# Autodesk Inventor assembly: printer
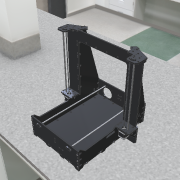
[picture p0: Inventor's stored thumbnail of the model, 180x180]
Saved by Autodesk Inventor 2014 (Build 180170000, 170)
## iProperties
Created: 2014-01-09
Part Number: printer
Document SubType Name: Assembly
Designer: buben
Author: buben
## Documents named in this file (21)
- C:\Users\buben\Documents\GitHub\bacon\inventor files\assemblies\printer.iam
- C:\Users\buben\Documents\GitHub\bacon\inventor files\printer parts\brace_left.ipt
- C:\Users\buben\Documents\GitHub\bacon\inventor files\printer parts\bottom.ipt
- C:\Users\buben\Documents\GitHub\bacon\inventor files\printer parts\brace_right.ipt
- C:\Users\buben\Documents\GitHub\bacon\inventor files\printer parts\front.ipt
- C:\Users\buben\Documents\GitHub\bacon\inventor files\printer parts\back.ipt
- C:\Users\buben\Documents\GitHub\bacon\inventor files\printer parts\frame.ipt
- C:\Users\buben\Documents\GitHub\bacon\inventor files\printer parts\z_motor_brace.ipt
- C:\Users\buben\Documents\GitHub\bacon\inventor files\printer parts\z_motor_mount.ipt
- C:\Users\buben\Documents\GitHub\bacon\inventor files\printer parts\y_axis_cap.ipt
- C:\Users\buben\Documents\GitHub\bacon\inventor files\printer parts\z_rod_stopper_bottom.ipt
- C:\Users\buben\Documents\GitHub\bacon\inventor files\3rd party components\nema_17_stepper\Imported Components\NEMA 17\NEMA 17.iam
- C:\Users\buben\Documents\GitHub\bacon\inventor files\utils\z_axis_rod.ipt
- C:\Users\buben\Documents\GitHub\bacon\inventor files\utils\z_threaded_rod.ipt
- C:\Users\buben\Documents\GitHub\bacon\inventor files\utils\y_axis_rod.ipt
- C:\Users\buben\Documents\GitHub\bacon\inventor files\printer parts\z_axis_top.ipt
- C:\Users\buben\Documents\GitHub\bacon\inventor files\printer parts\z_axis_top_cap.ipt
- C:\Users\buben\Documents\GitHub\bacon\inventor files\printer parts\frame_brace_top.ipt
- C:\Users\buben\Documents\GitHub\bacon\inventor files\utils\washer_m4.ipt
- C:\Users\buben\Documents\Inventor\Content Center Files\R2014\en-US\ISO 4762(2)\ISO 4762 - M4 x 20ISO.ipt
- C:\Users\buben\Documents\Inventor\Content Center Files\R2014\en-US\DIN 985\DIN 985 - M4.ipt
## Components (97 placed, 20 different names)
1. brace_left:1 — Mate:1, Mate:2, Mate:3, Mate:4, Mate:5, Flush:1, Mate:8, Mate:9, Mate:10, Mate:11, Mate:13, Mate:14, Mate:15, Mate:16, Mate:23, Mate:24, Mate:25, Mate:78, Mate:79, Mate:92
2. bottom:1 — Mate:4, Mate:5, Flush:1, Mate:6, Flush:2, Mate:7, Mate:12, Mate:74, Mate:80, Mate:91
3. brace_right:1 — Mate:6, Flush:2, Mate:7, Mate:26, Mate:28, Mate:70, Mate:72, Mate:73, Mate:90
4. front:1 — Mate:8, Mate:9, Mate:10, Mate:29, Mate:30, Mate:31, Mate:32, Mate:33, Mate:34, Mate:84, Mate:85, Mate:86, Mate:87, Mate:88, Mate:89
5. back:1 — Mate:11, Mate:12, Mate:13, Mate:35, Mate:36, Mate:37, Mate:38, Mate:39, Mate:40, Insert:3, Insert:4
6. frame:1 — Mate:14, Mate:15, Mate:16, Mate:17, Mate:18, Mate:19, Mate:20, Mate:21, Mate:22, Mate:27, Mate:57, Mate:58, Mate:59, Mate:60, Mate:61, Mate:62, Mate:69, Mate:71
7. z_motor_brace:1 — Mate:20, Mate:21, Mate:22
8. z_motor_brace:2 — Mate:17, Mate:18, Mate:19
9. z_motor_mount:1 — Mate:23, Mate:24, Mate:25, Mate:44, Mate:45, Mate:46, Mate:52, Insert:2
10. z_motor_mount:2 — Mate:26, Mate:27, Mate:28, Mate:41, Mate:42, Mate:43, Insert:1
11. y_axis_cap:1 — Mate:30, Mate:33, Mate:34
12. y_axis_cap:2 — Mate:35, Mate:39, Mate:40
13. y_axis_cap:3 — Mate:36, Mate:37, Mate:38
14. y_axis_cap:4 — Mate:29, Mate:31, Mate:32
15. z_rod_stopper_bottom:1 — Mate:44, Mate:45, Mate:46, Mate:50, Mate:51
16. z_rod_stopper_bottom:2 — Mate:41, Mate:42, Mate:43, Mate:47, Mate:48, Mate:49
17. NEMA 17:1 [sub-assembly] — Mate:47, Mate:48, Mate:49, Mate:53, Mate:54
18. NEMA 17:2 [sub-assembly] — Mate:50, Mate:51, Mate:52, Mate:55, Mate:56
19. z_axis_rod:1 — Insert:1
20. z_axis_rod:2 — Insert:2
21. z_threaded_rod:1 — Mate:55, Mate:56
22. z_threaded_rod:2 — Mate:53, Mate:54
23. y_axis_rod:1 — Insert:3
24. y_axis_rod:2 — Insert:4
25. z_axis_top:1 — Mate:57, Mate:58, Mate:59, Mate:63, Mate:67, Mate:68
26. z_axis_top:2 — Mate:60, Mate:61, Mate:62, Mate:64, Mate:65, Mate:66
27. z_axis_top_cap:1 — Mate:63, Mate:67, Mate:68
28. z_axis_top_cap:2 — Mate:64, Mate:65, Mate:66
29. frame_brace_top:1 — Mate:69, Mate:70, Mate:71
30. CSN 02 1702 B B 4,3:22 — Mate:86, Mate:87, Insert:8
31. CSN 02 1702 B B 4,3:25 — Mate:91, Mate:95, Mate:100
32. ISO 4762 M4 x 20:12 — Insert:8, Mate:95, Mate:101
33. DIN 985 - replaced by DIN EN ISO 10511 M4:11 — Mate:100, Mate:101
34. DIN 985 - replaced by DIN EN ISO 10511 M4:1 — Mate:76, Mate:77
35. CSN 02 1702 B B 4,3:2 — Mate:74, Mate:75, Mate:76
36. ISO 4762 M4 x 20:1 — Insert:5, Mate:75, Mate:77
37. CSN 02 1702 B B 4,3:1 — Mate:72, Mate:73, Insert:5
38. DIN 985 - replaced by DIN EN ISO 10511 M4:2
39. CSN 02 1702 B B 4,3:3
40. ISO 4762 M4 x 20:2
41. CSN 02 1702 B B 4,3:4
42. DIN 985 - replaced by DIN EN ISO 10511 M4:3
43. CSN 02 1702 B B 4,3:5
44. ISO 4762 M4 x 20:3
45. CSN 02 1702 B B 4,3:6
46. DIN 985 - replaced by DIN EN ISO 10511 M4:4
47. CSN 02 1702 B B 4,3:7
48. ISO 4762 M4 x 20:4
49. CSN 02 1702 B B 4,3:8
50. DIN 985 - replaced by DIN EN ISO 10511 M4:5
51. CSN 02 1702 B B 4,3:9
52. ISO 4762 M4 x 20:5
53. CSN 02 1702 B B 4,3:10
54. CSN 02 1702 B B 4,3:12 — Mate:78, Mate:79, Insert:6
55. ISO 4762 M4 x 20:6 — Insert:6, Mate:81, Mate:83
56. CSN 02 1702 B B 4,3:11 — Mate:80, Mate:81, Mate:82
57. DIN 985 - replaced by DIN EN ISO 10511 M4:6 — Mate:82, Mate:83
58. CSN 02 1702 B B 4,3:13
59. ISO 4762 M4 x 20:7
60. CSN 02 1702 B B 4,3:14
61. DIN 985 - replaced by DIN EN ISO 10511 M4:7
62. CSN 02 1702 B B 4,3:15
63. ISO 4762 M4 x 20:8
64. CSN 02 1702 B B 4,3:16
65. DIN 985 - replaced by DIN EN ISO 10511 M4:8
66. CSN 02 1702 B B 4,3:17
67. ISO 4762 M4 x 20:9
68. CSN 02 1702 B B 4,3:18
69. DIN 985 - replaced by DIN EN ISO 10511 M4:9
70. CSN 02 1702 B B 4,3:19
71. ISO 4762 M4 x 20:10
72. CSN 02 1702 B B 4,3:20
73. DIN 985 - replaced by DIN EN ISO 10511 M4:10
74. ISO 4762 M4 x 20:11 — Insert:7, Mate:94, Mate:97
75. CSN 02 1702 B B 4,3:21 — Mate:84, Mate:85, Insert:7
76. CSN 02 1702 B B 4,3:23 — Mate:90, Mate:94, Mate:96
77. DIN 985 - replaced by DIN EN ISO 10511 M4:13 — Mate:96, Mate:97
78. ISO 4762 M4 x 20:14
79. CSN 02 1702 B B 4,3:27
80. CSN 02 1702 B B 4,3:28
81. DIN 985 - replaced by DIN EN ISO 10511 M4:14
82. ISO 4762 M4 x 20:15
83. CSN 02 1702 B B 4,3:29
84. CSN 02 1702 B B 4,3:30
85. DIN 985 - replaced by DIN EN ISO 10511 M4:15
86. ISO 4762 M4 x 20:13 — Insert:9, Mate:93, Mate:99
87. CSN 02 1702 B B 4,3:24 — Mate:88, Mate:89, Insert:9
88. CSN 02 1702 B B 4,3:26 — Mate:92, Mate:93, Mate:98
89. DIN 985 - replaced by DIN EN ISO 10511 M4:12 — Mate:98, Mate:99
90. ISO 4762 M4 x 20:16
91. CSN 02 1702 B B 4,3:31
92. CSN 02 1702 B B 4,3:32
93. DIN 985 - replaced by DIN EN ISO 10511 M4:16
94. ISO 4762 M4 x 20:17
95. CSN 02 1702 B B 4,3:33
96. CSN 02 1702 B B 4,3:34
97. DIN 985 - replaced by DIN EN ISO 10511 M4:17
## Component patterns: (5 elements, first: DIN 985 - replaced by DIN EN ISO 10511 M4:1 + CSN 02 1702 B B 4,3:2 + ISO 4762 M4 x 20:1 + CSN 02 1702 B B 4,3:1), (5 elements, first: CSN 02 1702 B B 4,3:12 + ISO 4762 M4 x 20:6 + CSN 02 1702 B B 4,3:11 + DIN 985 - replaced by DIN EN ISO 10511 M4:6), (3 elements, first: ISO 4762 M4 x 20:11 + CSN 02 1702 B B 4,3:21 + CSN 02 1702 B B 4,3:23 + DIN 985 - replaced by DIN EN ISO 10511 M4:13), (3 elements, first: ISO 4762 M4 x 20:13 + CSN 02 1702 B B 4,3:24 + CSN 02 1702 B B 4,3:26 + DIN 985 - replaced by DIN EN ISO 10511 M4:12)
## Relationships (112: Mate 101, Insert 9, Flush 2)
- Mate:1: brace_left:1
- Mate:2: brace_left:1
- Mate:3: brace_left:1
- Mate:4: brace_left:1 ↔ bottom:1
- Mate:5: brace_left:1 ↔ bottom:1
- Flush:1: brace_left:1 ↔ bottom:1
- Mate:6: bottom:1 ↔ brace_right:1
- Flush:2: bottom:1 ↔ brace_right:1
- Mate:7: bottom:1 ↔ brace_right:1
- Mate:8: brace_left:1 ↔ front:1
- Mate:9: brace_left:1 ↔ front:1
- Mate:10: brace_left:1 ↔ front:1
- Mate:11: brace_left:1 ↔ back:1
- Mate:12: bottom:1 ↔ back:1
- Mate:13: brace_left:1 ↔ back:1
- Mate:14: brace_left:1 ↔ frame:1
- Mate:15: brace_left:1 ↔ frame:1
- Mate:16: brace_left:1 ↔ frame:1
- Mate:17: frame:1 ↔ z_motor_brace:2
- Mate:18: frame:1 ↔ z_motor_brace:2
- Mate:19: frame:1 ↔ z_motor_brace:2
- Mate:20: frame:1 ↔ z_motor_brace:1
- Mate:21: frame:1 ↔ z_motor_brace:1
- Mate:22: frame:1 ↔ z_motor_brace:1
- Mate:23: brace_left:1 ↔ z_motor_mount:1
- Mate:24: brace_left:1 ↔ z_motor_mount:1
- Mate:25: brace_left:1 ↔ z_motor_mount:1
- Mate:26: brace_right:1 ↔ z_motor_mount:2
- Mate:27: frame:1 ↔ z_motor_mount:2
- Mate:28: brace_right:1 ↔ z_motor_mount:2
- Mate:29: front:1 ↔ y_axis_cap:4
- Mate:30: front:1 ↔ y_axis_cap:1
- Mate:31: front:1 ↔ y_axis_cap:4
- Mate:32: front:1 ↔ y_axis_cap:4
- Mate:33: front:1 ↔ y_axis_cap:1
- Mate:34: front:1 ↔ y_axis_cap:1
- Mate:35: back:1 ↔ y_axis_cap:2
- Mate:36: back:1 ↔ y_axis_cap:3
- Mate:37: back:1 ↔ y_axis_cap:3
- Mate:38: back:1 ↔ y_axis_cap:3
- Mate:39: back:1 ↔ y_axis_cap:2
- Mate:40: back:1 ↔ y_axis_cap:2
- Mate:41: z_motor_mount:2 ↔ z_rod_stopper_bottom:2
- Mate:42: z_motor_mount:2 ↔ z_rod_stopper_bottom:2
- Mate:43: z_motor_mount:2 ↔ z_rod_stopper_bottom:2
- Mate:44: z_motor_mount:1 ↔ z_rod_stopper_bottom:1
- Mate:45: z_motor_mount:1 ↔ z_rod_stopper_bottom:1
- Mate:46: z_motor_mount:1 ↔ z_rod_stopper_bottom:1
- Mate:47: z_rod_stopper_bottom:2 ↔ NEMA 17:1
- Mate:48: z_rod_stopper_bottom:2 ↔ NEMA 17:1
- Mate:49: z_rod_stopper_bottom:2 ↔ NEMA 17:1
- Mate:50: z_rod_stopper_bottom:1 ↔ NEMA 17:2
- Mate:51: z_rod_stopper_bottom:1 ↔ NEMA 17:2
- Mate:52: z_motor_mount:1 ↔ NEMA 17:2
- Insert:1: z_motor_mount:2 ↔ z_axis_rod:1
- Insert:2: z_motor_mount:1 ↔ z_axis_rod:2
- Mate:53: NEMA 17:1 ↔ z_threaded_rod:2
- Mate:54: NEMA 17:1 ↔ z_threaded_rod:2
- Mate:55: NEMA 17:2 ↔ z_threaded_rod:1
- Mate:56: NEMA 17:2 ↔ z_threaded_rod:1
- Insert:3: back:1 ↔ y_axis_rod:1
- Insert:4: back:1 ↔ y_axis_rod:2
- Mate:57: frame:1 ↔ z_axis_top:1
- Mate:58: frame:1 ↔ z_axis_top:1
- Mate:59: frame:1 ↔ z_axis_top:1
- Mate:60: frame:1 ↔ z_axis_top:2
- Mate:61: frame:1 ↔ z_axis_top:2
- Mate:62: frame:1 ↔ z_axis_top:2
- Mate:63: z_axis_top:1 ↔ z_axis_top_cap:1
- Mate:64: z_axis_top:2 ↔ z_axis_top_cap:2
- Mate:65: z_axis_top:2 ↔ z_axis_top_cap:2
- Mate:66: z_axis_top:2 ↔ z_axis_top_cap:2
- Mate:67: z_axis_top:1 ↔ z_axis_top_cap:1
- Mate:68: z_axis_top:1 ↔ z_axis_top_cap:1
- Mate:69: frame:1 ↔ frame_brace_top:1
- Mate:70: brace_right:1 ↔ frame_brace_top:1
- Mate:71: frame:1 ↔ frame_brace_top:1
- Mate:72: brace_right:1 ↔ CSN 02 1702 B B 4,3:1
- Mate:73: brace_right:1 ↔ CSN 02 1702 B B 4,3:1
- Mate:74: bottom:1 ↔ CSN 02 1702 B B 4,3:2
- Insert:5: ISO 4762 M4 x 20:1 ↔ CSN 02 1702 B B 4,3:1
- Mate:75: CSN 02 1702 B B 4,3:2 ↔ ISO 4762 M4 x 20:1
- Mate:76: DIN 985 - replaced by DIN EN ISO 10511 M4:1 ↔ CSN 02 1702 B B 4,3:2
- Mate:77: DIN 985 - replaced by DIN EN ISO 10511 M4:1 ↔ ISO 4762 M4 x 20:1
- Mate:78: brace_left:1 ↔ CSN 02 1702 B B 4,3:12
- Mate:79: brace_left:1 ↔ CSN 02 1702 B B 4,3:12
- Mate:80: bottom:1 ↔ CSN 02 1702 B B 4,3:11
- Insert:6: CSN 02 1702 B B 4,3:12 ↔ ISO 4762 M4 x 20:6
- Mate:81: ISO 4762 M4 x 20:6 ↔ CSN 02 1702 B B 4,3:11
- Mate:82: CSN 02 1702 B B 4,3:11 ↔ DIN 985 - replaced by DIN EN ISO 10511 M4:6
- Mate:83: ISO 4762 M4 x 20:6 ↔ DIN 985 - replaced by DIN EN ISO 10511 M4:6
- Mate:84: front:1 ↔ CSN 02 1702 B B 4,3:21
- Mate:85: front:1 ↔ CSN 02 1702 B B 4,3:21
- Mate:86: front:1 ↔ CSN 02 1702 B B 4,3:22
- Mate:87: front:1 ↔ CSN 02 1702 B B 4,3:22
- Mate:88: front:1 ↔ CSN 02 1702 B B 4,3:24
- Mate:89: front:1 ↔ CSN 02 1702 B B 4,3:24
- Mate:90: brace_right:1 ↔ CSN 02 1702 B B 4,3:23
- Mate:91: bottom:1 ↔ CSN 02 1702 B B 4,3:25
- Mate:92: brace_left:1 ↔ CSN 02 1702 B B 4,3:26
- Insert:7: ISO 4762 M4 x 20:11 ↔ CSN 02 1702 B B 4,3:21
- Insert:8: CSN 02 1702 B B 4,3:22 ↔ ISO 4762 M4 x 20:12
- Insert:9: ISO 4762 M4 x 20:13 ↔ CSN 02 1702 B B 4,3:24
- Mate:93: ISO 4762 M4 x 20:13 ↔ CSN 02 1702 B B 4,3:26
- Mate:94: ISO 4762 M4 x 20:11 ↔ CSN 02 1702 B B 4,3:23
- Mate:95: CSN 02 1702 B B 4,3:25 ↔ ISO 4762 M4 x 20:12
- Mate:96: CSN 02 1702 B B 4,3:23 ↔ DIN 985 - replaced by DIN EN ISO 10511 M4:13
- Mate:97: ISO 4762 M4 x 20:11 ↔ DIN 985 - replaced by DIN EN ISO 10511 M4:13
- Mate:98: CSN 02 1702 B B 4,3:26 ↔ DIN 985 - replaced by DIN EN ISO 10511 M4:12
- Mate:99: ISO 4762 M4 x 20:13 ↔ DIN 985 - replaced by DIN EN ISO 10511 M4:12
- Mate:100: CSN 02 1702 B B 4,3:25 ↔ DIN 985 - replaced by DIN EN ISO 10511 M4:11
- Mate:101: ISO 4762 M4 x 20:12 ↔ DIN 985 - replaced by DIN EN ISO 10511 M4:11
